# Autodesk Inventor assembly: assemble
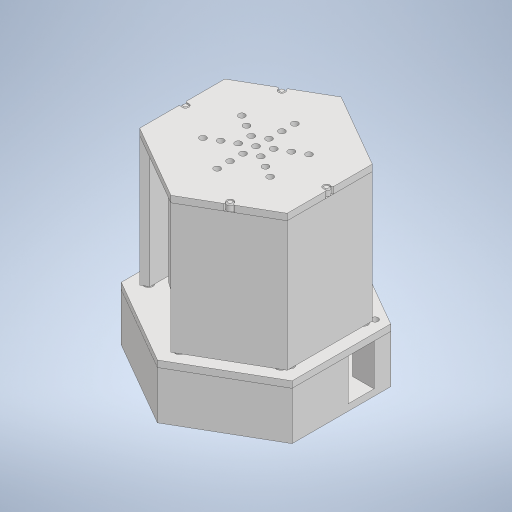
[picture p0: Inventor's stored thumbnail of the model, 512x512]
Saved by Autodesk Inventor 2024 (Build 280153000, 153)
## iProperties
Created: 2024-03-18
Part Number: assemble
Document SubType Name: Assembly
Designer: SSAFY
Author: SSAFY
## Documents named in this file (10)
- C:\Users\SSAFY\Desktop\TIL\3D\3D\2nd\assemble.iam
- C:\Users\SSAFY\Desktop\TIL\3D\3D\2nd\pi_case_bottom.ipt
- C:\Users\SSAFY\Desktop\TIL\3D\3D\2nd\pi_case_top.ipt
- C:\Users\SSAFY\Desktop\TIL\3D\3D\2nd\col.ipt
- C:\Users\SSAFY\Desktop\TIL\3D\3D\2nd\col_MIR.ipt
- C:\Users\SSAFY\Desktop\TIL\3D\3D\2nd\col_MIR1.ipt
- C:\Users\SSAFY\Desktop\TIL\3D\3D\2nd\inner_case_bottom.ipt
- C:\Users\SSAFY\Desktop\TIL\3D\3D\2nd\col_face.ipt
- C:\Users\SSAFY\Desktop\TIL\3D\3D\2nd\inner_top.ipt
- C:\Users\SSAFY\Desktop\TIL\3D\3D\2nd\top.ipt
## Components (15 placed, 9 different names)
1. pi_case_bottom:2 — 플러쉬:1, 플러쉬:2, 플러쉬:3, 메이트:1, 메이트:2, 메이트:4
2. pi_case_top:2 — 메이트:1, 메이트:2, 메이트:4, 메이트:5, 메이트:6, 메이트:7, 메이트:9, 메이트:10, 메이트:11, 메이트:13, 메이트:36, 메이트:37
3. col:1 — 메이트:5, 메이트:6, 메이트:7
4. col:2 — 메이트:9, 메이트:10, 메이트:11, 메이트:33, 메이트:34
5. col_MIR:1
6. col_MIR1:1 — 메이트:35, 메이트:36, 메이트:37
7. inner_case_bottom:1 — 메이트:13, 메이트:14, 메이트:15, 메이트:16, 메이트:17, 메이트:18, 메이트:19, 메이트:20, 메이트:21, 메이트:22, 메이트:23, 메이트:24, 메이트:25, 메이트:26
8. col_face:1 — 메이트:15, 메이트:16, 메이트:27, 메이트:28
9. col_face:2 — 메이트:19, 메이트:20
10. col_face:3 — 메이트:17, 메이트:18
11. col_face:4 — 메이트:23, 메이트:24
12. col_face:5 — 메이트:21, 메이트:22
13. col_face:6 — 메이트:25, 메이트:26
14. inner_top:1 — 메이트:27, 메이트:28
15. top:1 — 메이트:33, 메이트:34, 메이트:35
## Relationships (33: Mate 30, Flush 3)
- 플러쉬:1 [Flush]: pi_case_bottom:2
- 플러쉬:2 [Flush]: pi_case_bottom:2
- 플러쉬:3 [Flush]: pi_case_bottom:2
- 메이트:1 [Mate]: pi_case_bottom:2 ↔ pi_case_top:2
- 메이트:2 [Mate]: pi_case_bottom:2 ↔ pi_case_top:2
- 메이트:4 [Mate]: pi_case_bottom:2 ↔ pi_case_top:2
- 메이트:5 [Mate]: pi_case_top:2 ↔ col:1
- 메이트:6 [Mate]: pi_case_top:2 ↔ col:1
- 메이트:7 [Mate]: pi_case_top:2 ↔ col:1
- 메이트:9 [Mate]: pi_case_top:2 ↔ col:2
- 메이트:10 [Mate]: pi_case_top:2 ↔ col:2
- 메이트:11 [Mate]: pi_case_top:2 ↔ col:2
- 메이트:13 [Mate] (4 mm): pi_case_top:2 ↔ inner_case_bottom:1
- 메이트:14 [Mate]: inner_case_bottom:1
- 메이트:15 [Mate]: inner_case_bottom:1 ↔ col_face:1
- 메이트:16 [Mate]: inner_case_bottom:1 ↔ col_face:1
- 메이트:17 [Mate]: inner_case_bottom:1 ↔ col_face:3
- 메이트:18 [Mate]: inner_case_bottom:1 ↔ col_face:3
- 메이트:19 [Mate]: inner_case_bottom:1 ↔ col_face:2
- 메이트:20 [Mate]: inner_case_bottom:1 ↔ col_face:2
- 메이트:21 [Mate]: inner_case_bottom:1 ↔ col_face:5
- 메이트:22 [Mate]: inner_case_bottom:1 ↔ col_face:5
- 메이트:23 [Mate]: inner_case_bottom:1 ↔ col_face:4
- 메이트:24 [Mate]: inner_case_bottom:1 ↔ col_face:4
- 메이트:25 [Mate]: inner_case_bottom:1 ↔ col_face:6
- 메이트:26 [Mate]: inner_case_bottom:1 ↔ col_face:6
- 메이트:27 [Mate]: col_face:1 ↔ inner_top:1
- 메이트:28 [Mate]: col_face:1 ↔ inner_top:1
- 메이트:33 [Mate]: col:2 ↔ top:1
- 메이트:34 [Mate]: col:2 ↔ top:1
- 메이트:35 [Mate]: col_MIR1:1 ↔ top:1
- 메이트:36 [Mate]: pi_case_top:2 ↔ col_MIR1:1
- 메이트:37 [Mate]: pi_case_top:2 ↔ col_MIR1:1
